# Autodesk Inventor assembly: Complete Thumb
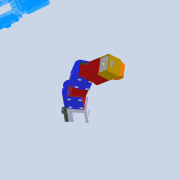
[picture p0: Inventor's stored thumbnail of the model, 180x180]
Saved by Autodesk Inventor 2020 (Build 240168000, 168)
## iProperties
Created: 2020-02-17
Part Number: Complete Thumb
Document SubType Name: Assembly
Designer: PROXS
Author: PROXS
## Documents named in this file (4)
- C:\Users\sami_\Documents\V1.6\Workgroups\NotInProject\THUMB\Assembly\Complete Thumb.iam
- C:\Users\sami_\Documents\V1.6\Workgroups\NotInProject\THUMB\Assembly\Tip.iam
- C:\Users\sami_\Documents\V1.6\thumbL2.iam
- C:\Users\sami_\Documents\V1.6\ThumbL3.iam
## Components (3 placed, 3 different names)
1. thumbL2:1 [sub-assembly]
2. ThumbL3:1 [sub-assembly]
3. Tip:1 [sub-assembly]
## Relationships (4: RevoluteJoint 2, Mate 2)
- [RevoluteJoint]: thumbL2:1 ↔ ThumbL3:1
- [RevoluteJoint]: ThumbL3:1 ↔ Tip:1
- [Mate]: ThumbL3:1 ↔ Tip:1
- [Mate]: thumbL2:1 ↔ ThumbL3:1
